# Autodesk Inventor assembly: WKA
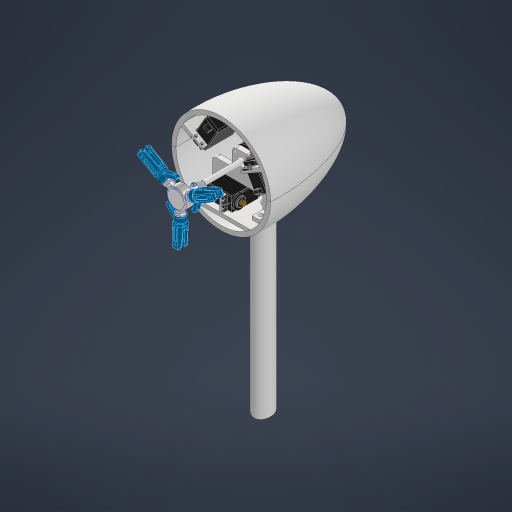
[picture p0: Inventor's stored thumbnail of the model, 512x512]
Saved by Autodesk Inventor 2023.2 (Build 272271000, 271)
## iProperties
Created: 2023-04-13
Part Number: WKA
Document SubType Name: Assembly
Designer: tadeus
Author: tadeus
## Documents named in this file (6)
- C:\Users\tadeu\Documents\0 Nerdy\CAD\Inventor\Studium\5. Semester\NWPL\WKA\Bauteile\WKA.iam
- C:\Users\tadeu\Documents\0 Nerdy\CAD\Inventor\Studium\5. Semester\NWPL\WKA\Bauteile\Gehäuse\Gehäuse.ipt
- C:\Users\tadeu\Documents\0 Nerdy\CAD\Inventor\Studium\5. Semester\NWPL\WKA\Bauteile\Rotorkopf\Rotrkopf.iam
- C:\Users\tadeu\Documents\0 Nerdy\CAD\Inventor\Studium\5. Semester\NWPL\WKA\Bauteile\Technik\Servo\Servo.iam
- C:\Users\tadeu\Documents\0 Nerdy\CAD\Inventor\Studium\5. Semester\NWPL\WKA\Bauteile\Gehäuse\Bracket vorne.ipt
- C:\Users\tadeu\Documents\0 Nerdy\CAD\Inventor\Studium\5. Semester\NWPL\WKA\Bauteile\Gehäuse\Bracket hinten.ipt
## Components (7 placed, 5 different names)
1. Gehäuse:1 — Einfügen:1, Einfügen:2, Einfügen:3, Einfügen:4
2. Rotrkopf:1 [sub-assembly] — Einfügen:5, Einfügen:6
3. Servo:1 [sub-assembly] — Einfügen:1
4. Servo:2 [sub-assembly] — Einfügen:2
5. Servo:3 [sub-assembly] — Einfügen:3
6. Bracket vorne:1 — Einfügen:4, Einfügen:5
7. Bracket hinten:1 — Einfügen:6
## Relationships (6: Insert 6)
- Einfügen:1 [Insert]: Gehäuse:1 ↔ Servo:1
- Einfügen:2 [Insert]: Gehäuse:1 ↔ Servo:2
- Einfügen:3 [Insert]: Gehäuse:1 ↔ Servo:3
- Einfügen:4 [Insert]: Gehäuse:1 ↔ Bracket vorne:1
- Einfügen:5 [Insert]: Rotrkopf:1 ↔ Bracket vorne:1
- Einfügen:6 [Insert]: Rotrkopf:1 ↔ Bracket hinten:1
